# Autodesk Inventor assembly: zlozenie
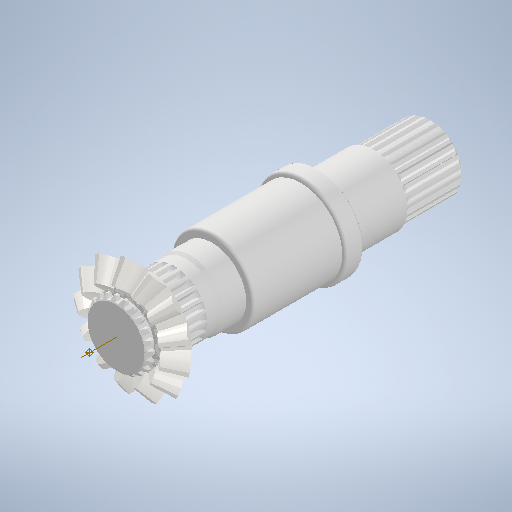
[picture p0: Inventor's stored thumbnail of the model, 512x512]
Saved by Autodesk Inventor 2025.2 (Build 292293000, 293)
## iProperties
Created: 2025-06-10
Part Number: zlozenie
Document SubType Name: Assembly
Designer: Kacper
Author: Kacper
## Documents named in this file (3)
- D:\studia\semestr 4\Grafika inżynierska\Projekt 4\zlozenie.iam
- D:\studia\semestr 4\Grafika inżynierska\Projekt 4\shaft.ipt
- D:\studia\semestr 4\Grafika inżynierska\Projekt 4\gear_base.ipt
## Components (2 placed, 2 different names)
1. shaft:1 — Mate:1, Flush:1
2. Bevel Gear1:1 — Mate:1, Flush:1
## Relationships (2: Mate 1, Flush 1)
- Mate:1: shaft:1 ↔ Bevel Gear1:1
- Flush:1: shaft:1 ↔ Bevel Gear1:1
